# Autodesk Inventor assembly: 6082RS
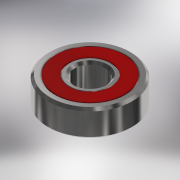
[picture p0: Inventor's stored thumbnail of the model, 180x180]
Saved by Autodesk Inventor 2017 (Build 210142000, 142)
## iProperties
Created: 2016-08-26
Part Number: 6082RS
Document SubType Name: Assembly
Designer: Ali
Author: Ali
## Documents named in this file (3)
- C:\Users\Ali\Dropbox\Work\Project\Inventor\Parts\6082RS.iam
- C:\Users\Ali\Dropbox\Work\Project\Inventor\Parts\608-outer.ipt
- C:\Users\Ali\Dropbox\Work\Project\Inventor\Parts\608-inner.ipt
## Components (2 placed, 2 different names)
1. 608-outer:1 — Flush:1
2. 608-inner:1 — Flush:1
## Relationships (1: Flush 1)
- Flush:1: 608-outer:1 ↔ 608-inner:1
